# Autodesk Inventor assembly: Zespół1
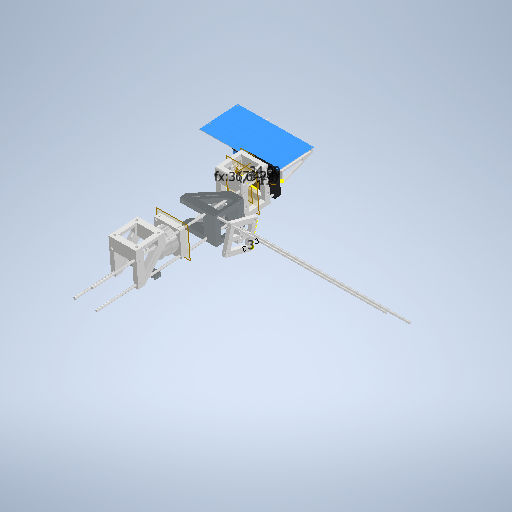
[picture p0: Inventor's stored thumbnail of the model, 512x512]
Saved by Autodesk Inventor 2025.1 (Build 291241000, 241)
## iProperties
Created: 2024-10-25
Part Number: Zespół1
Document SubType Name: Assembly
Designer: PC
Author: PC
## Documents named in this file (17)
- C:\Users\PC\Desktop\fotolito_czesci\nowe\main.iam
- C:\Users\PC\Desktop\fotolito_czesci\nowe\plyta_dmd.iam
- electronics_assembly.iam
- C:\Users\PC\Desktop\fotolito_czesci\rod.ipt
- C:\Users\PC\Desktop\fotolito_czesci\nowe\wyliczenia.ipt
- C:\Users\PC\Desktop\fotolito_czesci\nowe\6_2xclamp_back.ipt
- C:\Users\PC\Desktop\fotolito_czesci\nowe\6_2xclamp_main.ipt
- C:\Users\PC\Desktop\fotolito_czesci\nowe\wzmocnienie.ipt
- C:\Users\PC\Desktop\fotolito_czesci\nowe\genera_ mount.ipt
- C:\Users\PC\Desktop\fotolito_czesci\nowe\beamsplitter.ipt
- C:\Users\PC\Desktop\fotolito_czesci\nowe\camera_60mm.ipt
- C:\Users\PC\Desktop\fotolito_czesci\nowe\6xMounting_base.ipt
- C:\Users\PC\Desktop\fotolito_czesci\nowe\6xMounting_clamp.ipt
- C:\Users\PC\Desktop\fotolito_czesci\nowe\beamsplitter_mirror.ipt
- C:\Users\PC\Desktop\fotolito_czesci\nowe\iluminator.ipt
- C:\Users\PC\Desktop\output\mirror_recepticle.ipt
- C:\Users\PC\Desktop\fotolito_czesci\nowe\obiektyw.ipt
## Components (24 placed, 15 different names)
1. electronics_assembly:1 [sub-assembly] — Zestawiające:2, Zestawiające:3, Zestawiające:4, Zestawiające:5, Zestawiające:6, Równoległe:2, Zestawiające:8, Zestawiające:9, Zestawiające:12, Zestawiające:14, Zestawiające:16, Zestawiające:19, Zestawiające:21, Równoległe:3, Równoległe:6, Równoległe:14, Zestawiające:60, Zestawiające:61
2. rod:3 — Zestawiające:3, Zestawiające:5, Zestawiające:41, Symetria:1, Zestawiające:49, Zestawiające:56
3. rod:4 — Zestawiające:4, Równoległe:2, Symetria:1, Zestawiające:44, Zestawiające:63, Zestawiające:66
4. rod:2 — Zestawiające:2, Zestawiające:6, Zestawiające:23, Zestawiające:25, Zestawiające:45, Zestawiające:50, Zestawiające:51, Zestawiające:55, Zestawiające:62, Zestawiające:67
5. wyliczenia:1 — Zestawiające:8, Zestawiające:9, Zestawiające:11, Kątowe:2, Kątowe:3, Zestawiające:13, Kątowe:4, Kątowe:5, Zestawiające:15, Kątowe:6, Kątowe:7, Zestawiające:17, Kątowe:8, Zestawiające:18, Kątowe:9, Kątowe:10, Zestawiające:26, Zestawiające:27, Równoległe:5, Zestawiające:58, Zestawiające:59, Równoległe:16
6. rod:5 — Zestawiające:21, Równoległe:3, Zestawiające:22, Zestawiające:24, Zestawiające:40
7. 6_2xclamp_back:1 — Zestawiające:24, Zestawiające:25, Równoległe:4
8. 6_2xclamp_main:1 — Zestawiające:22, Zestawiające:23, Równoległe:4, Zestawiające:26, Zestawiające:27, Równoległe:5
9. wzmocnienie:1 — Równoległe:7, Równoległe:9
10. rod:6 — Równoległe:12, Zestawiające:46, Zestawiające:48
11. rod:7 — Równoległe:12, Zestawiające:47
12. genera_ mount:1 — Zestawiające:40, Zestawiające:41
13. beamsplitter:1 — Zestawiające:44, Zestawiające:45, Zestawiające:46, Zestawiające:47, Zestawiające:53, Zestawiające:57, Równoległe:13
14. camera_60mm:1 — Zestawiające:48
15. 6xMounting_base:1 — Zestawiające:49, Zestawiające:50, Zestawiające:52
16. 6xMounting_clamp:1 — Zestawiające:51, Zestawiające:52
17. beamsplitter_mirror:1 — Zestawiające:53, Zestawiające:57, Równoległe:13
18. 6xMounting_base:2 — Zestawiające:55, Zestawiające:56
19. 6xMounting_clamp:2
20. iluminator:1 — Równoległe:14, Równoległe:15
21. mirror_recepticle:1 — Równoległe:15, Równoległe:16, Zestawiające:60, Zestawiające:61
22. genera_ mount:2 — Zestawiające:62, Zestawiające:63, Zestawiające:64, Zestawiające:65
23. obiektyw:1 — Zestawiające:64, Zestawiające:65
24. beamsplitter:2 — Zestawiające:66, Zestawiające:67
## Relationships (71: Mate 49, Flush 12, Angle 9, Symmetry 1)
- Zestawiające:2 [Mate]: electronics_assembly:1 ↔ rod:2
- Zestawiające:3 [Mate]: electronics_assembly:1 ↔ rod:3
- Zestawiające:4 [Mate]: electronics_assembly:1 ↔ rod:4
- Zestawiające:5 [Mate]: electronics_assembly:1 ↔ rod:3
- Zestawiające:6 [Mate]: electronics_assembly:1 ↔ rod:2
- Równoległe:2 [Flush]: electronics_assembly:1 ↔ rod:4
- Zestawiające:8 [Mate]: electronics_assembly:1 ↔ wyliczenia:1
- Zestawiające:9 [Mate]: electronics_assembly:1 ↔ wyliczenia:1
- Zestawiające:11 [Mate]: wyliczenia:1
- Kątowe:2 [Angle] (0 deg): wyliczenia:1
- Zestawiające:12 [Mate]: electronics_assembly:1
- Kątowe:3 [Angle] (0 deg): wyliczenia:1
- Zestawiające:13 [Mate]: wyliczenia:1
- Kątowe:4 [Angle] (0 deg): wyliczenia:1
- Zestawiające:14 [Mate]: electronics_assembly:1
- Kątowe:5 [Angle] (0 deg): wyliczenia:1
- Zestawiające:15 [Mate]: wyliczenia:1
- Kątowe:6 [Angle] (0 deg): wyliczenia:1
- Zestawiające:16 [Mate]: electronics_assembly:1
- Kątowe:7 [Angle] (0 deg): wyliczenia:1
- Zestawiające:17 [Mate]: wyliczenia:1
- Kątowe:8 [Angle] (0 deg): wyliczenia:1
- Zestawiające:18 [Mate]: wyliczenia:1
- Kątowe:9 [Angle] (0 deg): wyliczenia:1
- Zestawiające:19 [Mate]: electronics_assembly:1
- Kątowe:10 [Angle] (0 deg): wyliczenia:1
- Zestawiające:21 [Mate]: electronics_assembly:1 ↔ rod:5
- Równoległe:3 [Flush]: electronics_assembly:1 ↔ rod:5
- Zestawiające:22 [Mate]: rod:5 ↔ 6_2xclamp_main:1
- Zestawiające:23 [Mate]: rod:2 ↔ 6_2xclamp_main:1
- Zestawiające:24 [Mate]: rod:5 ↔ 6_2xclamp_back:1
- Zestawiające:25 [Mate]: rod:2 ↔ 6_2xclamp_back:1
- Równoległe:4 [Flush]: 6_2xclamp_back:1 ↔ 6_2xclamp_main:1
- Zestawiające:26 [Mate]: wyliczenia:1 ↔ 6_2xclamp_main:1
- Zestawiające:27 [Mate]: wyliczenia:1 ↔ 6_2xclamp_main:1
- Równoległe:5 [Flush]: wyliczenia:1 ↔ 6_2xclamp_main:1
- Równoległe:6 [Flush] (7.5 mm): electronics_assembly:1
- Równoległe:7 [Flush]: wzmocnienie:1
- Równoległe:9 [Flush]: wzmocnienie:1
- Równoległe:12 [Flush]: rod:6 ↔ rod:7
- Zestawiające:40 [Mate]: rod:5 ↔ genera_ mount:1
- Zestawiające:41 [Mate]: rod:3 ↔ genera_ mount:1
- Symetria:1 [Symmetry]: rod:3 ↔ rod:4
- Zestawiające:44 [Mate]: rod:4 ↔ beamsplitter:1
- Zestawiające:45 [Mate]: rod:2 ↔ beamsplitter:1
- Zestawiające:46 [Mate]: rod:6 ↔ beamsplitter:1
- Zestawiające:47 [Mate]: rod:7 ↔ beamsplitter:1
- Zestawiające:48 [Mate]: rod:6 ↔ camera_60mm:1
- Zestawiające:49 [Mate]: rod:3 ↔ 6xMounting_base:1
- Zestawiające:50 [Mate]: rod:2 ↔ 6xMounting_base:1
- Zestawiające:51 [Mate]: rod:2 ↔ 6xMounting_clamp:1
- Zestawiające:52 [Mate]: 6xMounting_base:1 ↔ 6xMounting_clamp:1
- Zestawiające:53 [Mate]: beamsplitter:1 ↔ beamsplitter_mirror:1
- [Mate]: 6xMounting_base:2 ↔ 6xMounting_clamp:2
- Zestawiające:55 [Mate]: rod:2 ↔ 6xMounting_base:2
- Zestawiające:56 [Mate]: rod:3 ↔ 6xMounting_base:2
- Zestawiające:57 [Mate]: beamsplitter:1 ↔ beamsplitter_mirror:1
- Równoległe:13 [Flush]: beamsplitter:1 ↔ beamsplitter_mirror:1
- Równoległe:14 [Flush]: electronics_assembly:1 ↔ iluminator:1
- Zestawiające:58 [Mate]: wyliczenia:1
- Zestawiające:59 [Mate]: wyliczenia:1
- Równoległe:15 [Flush]: iluminator:1 ↔ mirror_recepticle:1
- Równoległe:16 [Flush]: wyliczenia:1 ↔ mirror_recepticle:1
- Zestawiające:60 [Mate]: electronics_assembly:1 ↔ mirror_recepticle:1
- Zestawiające:61 [Mate]: electronics_assembly:1 ↔ mirror_recepticle:1
- Zestawiające:62 [Mate]: rod:2 ↔ genera_ mount:2
- Zestawiające:63 [Mate]: rod:4 ↔ genera_ mount:2
- Zestawiające:64 [Mate]: genera_ mount:2 ↔ obiektyw:1
- Zestawiające:65 [Mate]: genera_ mount:2 ↔ obiektyw:1
- Zestawiające:66 [Mate]: rod:4 ↔ beamsplitter:2
- Zestawiające:67 [Mate]: rod:2 ↔ beamsplitter:2
## Named parameters: d94_d92 = 0 mm, Finish1_Area = 444.409, Finish1_Thickness = 0.05 mm, Finish2_Area = 376.991, Finish3_Area = 188.496
note: some values were not read from the file. Shown as the stored number, unit unknown: "Finish1_Area", "Finish2_Area", "Finish3_Area".
